# Autodesk Inventor assembly: Link1
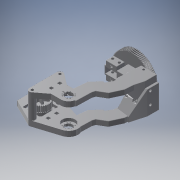
[picture p0: Inventor's stored thumbnail of the model, 180x180]
Saved by Autodesk Inventor 2019 (Build 230136000, 136)
## iProperties
Created: 2020-02-16
Part Number: Link1
Document SubType Name: Assembly
Designer: Alex
Author: Alex
## Documents named in this file (6)
- D:\Alex\Documents\GitHub\RBE3001-URDF-Example\STLs\FinalSTLS\Inventor_Assy\Link1.iam
- D:\Alex\Documents\Personal Projects\BenchPowerSupply\0_Link_baseEncoderCap0_limb_0_Part_5.ipt
- D:\Alex\Documents\Personal Projects\BenchPowerSupply\0_Link_drivenGear_limb_0_Part_7.ipt
- D:\Alex\Documents\Personal Projects\BenchPowerSupply\0_Link_loadCellBlock_limb_0_Part_6.ipt
- D:\Alex\Documents\Personal Projects\BenchPowerSupply\0_Link_servoGear_limb_0_Part_0.ipt
- D:\Alex\Documents\Personal Projects\BenchPowerSupply\0_Link_sidePlate0_limb_0_Part_4.ipt
## Components (5 placed, 5 different names)
1. 0_Link_baseEncoderCap0_limb_0_Part_5:1 — Flush:1, Flush:2, Flush:3
2. 0_Link_sidePlate0_limb_0_Part_4:1 — Flush:4, Flush:5, Flush:6
3. 0_Link_drivenGear_limb_0_Part_7:1 — Flush:7, Flush:8, Flush:9
4. 0_Link_loadCellBlock_limb_0_Part_6:1 — Flush:13, Flush:14, Flush:15
5. 0_Link_servoGear_limb_0_Part_0:1 — Flush:16, Flush:17, Flush:18
## Relationships (15: Flush 15)
- Flush:1: 0_Link_baseEncoderCap0_limb_0_Part_5:1
- Flush:2: 0_Link_baseEncoderCap0_limb_0_Part_5:1
- Flush:3: 0_Link_baseEncoderCap0_limb_0_Part_5:1
- Flush:4: 0_Link_sidePlate0_limb_0_Part_4:1
- Flush:5: 0_Link_sidePlate0_limb_0_Part_4:1
- Flush:6: 0_Link_sidePlate0_limb_0_Part_4:1
- Flush:7: 0_Link_drivenGear_limb_0_Part_7:1
- Flush:8: 0_Link_drivenGear_limb_0_Part_7:1
- Flush:9: 0_Link_drivenGear_limb_0_Part_7:1
- Flush:13: 0_Link_loadCellBlock_limb_0_Part_6:1
- Flush:14: 0_Link_loadCellBlock_limb_0_Part_6:1
- Flush:15: 0_Link_loadCellBlock_limb_0_Part_6:1
- Flush:16: 0_Link_servoGear_limb_0_Part_0:1
- Flush:17: 0_Link_servoGear_limb_0_Part_0:1
- Flush:18: 0_Link_servoGear_limb_0_Part_0:1
